# Autodesk Inventor assembly: MontagemComPosicionamento
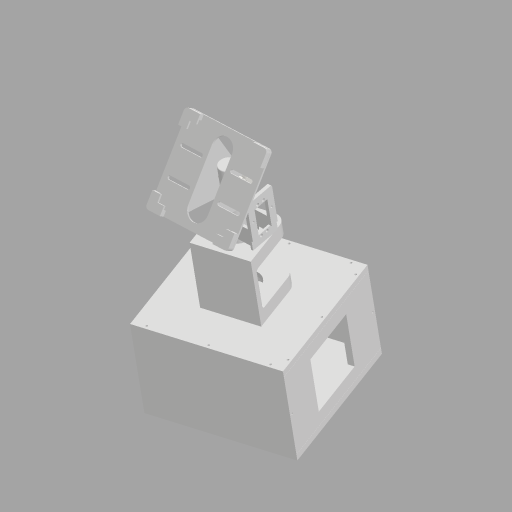
[picture p0: Inventor's stored thumbnail of the model, 512x512]
Saved by Autodesk Inventor 2023.2 (Build 272271030, 271C)
## iProperties
Created: 2024-06-18
Part Number: MontagemComPosicionamento
Document SubType Name: Assembly
Designer: VICTOR
Author: VICTOR
## Documents named in this file (12)
- C:\Users\VICTOR\OneDrive\Área de Trabalho\TCC_Final\modelagem3D\modelosCAD\MontagemComPosicionamento.iam
- C:\Users\VICTOR\OneDrive\Área de Trabalho\TCC_Final\modelagem3D\modelosCAD\BaseEncima.ipt
- C:\Users\VICTOR\OneDrive\Área de Trabalho\TCC_Final\modelagem3D\modelosCAD\Lateral.ipt
- C:\Users\VICTOR\OneDrive\Área de Trabalho\TCC_Final\modelagem3D\modelosCAD\Lateral1-2.ipt
- C:\Users\VICTOR\OneDrive\Área de Trabalho\TCC_Final\modelagem3D\modelosCAD\BaseEmbaixoFuros.ipt
- C:\Users\VICTOR\OneDrive\Área de Trabalho\TCC_Final\modelagem3D\modelosCAD\eixo_6_193_5_249_motor_furo99_2.ipt
- C:\Users\VICTOR\OneDrive\Área de Trabalho\TCC_Final\modelagem3D\modelosCAD\engrenagem16_45_69.ipt
- C:\Users\VICTOR\OneDrive\Área de Trabalho\TCC_Final\modelagem3D\modelosCAD\Part1_Movel_30_60_largo_7mm.ipt
- C:\Users\VICTOR\OneDrive\Área de Trabalho\TCC_Final\modelagem3D\modelosCAD\ApoioBaseCilindrica47_5.ipt
- C:\Users\VICTOR\OneDrive\Área de Trabalho\TCC_Final\modelagem3D\modelosCAD\MG995_apoio.ipt
- C:\Users\VICTOR\OneDrive\Área de Trabalho\TCC_Final\modelagem3D\modelosCAD\MG995_26_apoio_upgrade.ipt
- C:\Users\VICTOR\OneDrive\Área de Trabalho\TCC_Final\modelagem3D\modelosCAD\PresasPlaca_4.ipt
## Components (15 placed, 11 different names)
1. BaseEncima:1 — Rigid:1, Rotational:1, Rigid:5
2. Lateral:1 — Rigid:1, Rigid:2, Rigid:3, Mate:1
3. Lateral1-2:1 — Rigid:2
4. Lateral1-2:2 — Rigid:3
5. BaseEmbaixoFuros:1 — Mate:1
6. eixo_6_193_5_249_motor_furo99_2:1 — Rotational:1, Rotational:2, Rigid:6
7. Part1_Movel_30_60_largo_7mm:1 — Rigid:4, Rigid:8, Rigid:9, Rigid:10, Rigid:11
8. Spur Gear2:2 — Rigid:4, Rotational:2
9. ApoioBaseCilindrica47_5:1 — Rigid:5
10. MG995_apoio:1 — Rigid:6, Rigid:7
11. MG995_26_apoio_upgrade:1 — Rigid:7
12. PresasPlaca_4:4 — Rigid:8
13. PresasPlaca_4:5 — Rigid:9
14. PresasPlaca_4:6 — Rigid:10
15. PresasPlaca_4:7 — Rigid:11
## Relationships (14: WeldJoint 11, RevoluteJoint 2, Mate 1)
- Rigid:1 [WeldJoint]: BaseEncima:1 ↔ Lateral:1
- Rigid:2 [WeldJoint]: Lateral:1 ↔ Lateral1-2:1
- Rigid:3 [WeldJoint]: Lateral:1 ↔ Lateral1-2:2
- Mate:1: Lateral:1 ↔ BaseEmbaixoFuros:1
- Rotational:1 [RevoluteJoint]: BaseEncima:1 ↔ eixo_6_193_5_249_motor_furo99_2:1
- Rigid:4 [WeldJoint]: Part1_Movel_30_60_largo_7mm:1 ↔ Spur Gear2:2
- Rotational:2 [RevoluteJoint]: eixo_6_193_5_249_motor_furo99_2:1 ↔ Spur Gear2:2
- Rigid:5 [WeldJoint]: BaseEncima:1 ↔ ApoioBaseCilindrica47_5:1
- Rigid:6 [WeldJoint]: eixo_6_193_5_249_motor_furo99_2:1 ↔ MG995_apoio:1
- Rigid:7 [WeldJoint]: MG995_apoio:1 ↔ MG995_26_apoio_upgrade:1
- Rigid:8 [WeldJoint]: Part1_Movel_30_60_largo_7mm:1 ↔ PresasPlaca_4:4
- Rigid:9 [WeldJoint]: Part1_Movel_30_60_largo_7mm:1 ↔ PresasPlaca_4:5
- Rigid:10 [WeldJoint]: Part1_Movel_30_60_largo_7mm:1 ↔ PresasPlaca_4:6
- Rigid:11 [WeldJoint]: Part1_Movel_30_60_largo_7mm:1 ↔ PresasPlaca_4:7
